# Autodesk Inventor assembly: Toughbox Mini
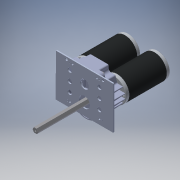
[picture p0: Inventor's stored thumbnail of the model, 180x180]
Saved by Autodesk Inventor 2016 (Build 200138000, 138)
## iProperties
Created: 2016-01-25
Part Number: Toughbox Mini
Document SubType Name: Assembly
Designer: Mentor1102
Author: Mentor1102
Revision Number: ANY
## Documents named in this file (8)
- C:\Users\Mentor1102\Desktop\5632 CAD\Toughbox Mini.iam
- C:\Users\Mentor1102\Downloads\10-32 Nylock Nut.ipt
- C:\Users\Mentor1102\Downloads\TM Housing.ipt
- C:\Users\Mentor1102\Downloads\SHCS 10-32 x 0.625.ipt
- C:\Users\Mentor1102\Downloads\R6ZZ Bearing.ipt
- C:\Users\Mentor1102\Desktop\5632 CAD\TM Flat Shaft Plate.ipt
- C:\Users\Mentor1102\Desktop\5632 CAD\CIM Motor SW.ipt
- C:\Users\Mentor1102\Downloads\AM-0396_LONG_TOUGHBOX_HEX_S_AF3.ipt
## Components (14 placed, 13 different names)
1. 10-32 Nylock Nut_74
2. 10-32 Nylock Nut_75
3. 10-32 Nylock Nut_76
4. 10-32 Nylock Nut_77
5. TM Housing_84 — Mate:1, Mate:2, Insert:2, Insert:3, Insert:4
6. SHCS 10-32 x 0.625_85
7. SHCS 10-32 x 0.625_91
8. SHCS 10-32 x 0.625_92
9. R6ZZ Bearing_93
10. R6ZZ Bearing_94
11. TM Flat Shaft Plate:1 — Mate:1, Mate:2
12. CIM Motor SW:1 — Insert:2
13. CIM Motor SW:2 — Insert:3
14. AM-0396_LONG_TOUGHBOX_HEX_S_AF3:1 — Insert:4
## Relationships (5: Insert 3, Mate 2)
- Mate:1: TM Housing_84 ↔ TM Flat Shaft Plate:1
- Mate:2: TM Housing_84 ↔ TM Flat Shaft Plate:1
- Insert:2: TM Housing_84 ↔ CIM Motor SW:1
- Insert:3: TM Housing_84 ↔ CIM Motor SW:2
- Insert:4: TM Housing_84 ↔ AM-0396_LONG_TOUGHBOX_HEX_S_AF3:1
